# Autodesk Inventor assembly: ENSAMBLE CUERPO M 2020-9.5L
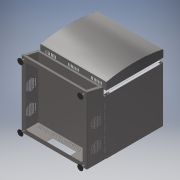
[picture p0: Inventor's stored thumbnail of the model, 180x180]
Saved by Autodesk Inventor 2017 (Build 210142000, 142)
## iProperties
Created: 2021-02-12
Part Number: ENSAMBLE CUERPO M 2020-9.5L
Description: STEP AP214
Document SubType Name: Assembly
Designer: USUARIO
Sending System: SolidWorks 2013
Preprocessor: SwSTEP 2.0
Title: ENSAMBLE CUERPO M 2020-9.5L.STEP
Revision Number: ANY
## Documents named in this file (10)
- D:\Laboratorio\Mufla\2021\Mufla 9L Psoc Artilab #0045884XX OP202139\Modelo\ENSAMBLE CUERPO M 2020-9.5L.iam
- D:\Laboratorio\Mufla\2021\Mufla 9L Psoc Artilab #0045884XX OP202139\Modelo\BASE M 2019-9.5L.ipt
- D:\Laboratorio\Mufla\2021\Mufla 9L Psoc Artilab #0045884XX OP202139\Modelo\TUERCA REMACHABLE 0,3125.ipt
- D:\Laboratorio\Mufla\2021\Mufla 9L Psoc Artilab #0045884XX OP202139\Modelo\PATA 5-16.ipt
- D:\Laboratorio\Mufla\2021\Mufla 9L Psoc Artilab #0045884XX OP202139\Modelo\RESPIRADERO M2018-2.2L.ipt
- D:\Laboratorio\Mufla\2021\Mufla 9L Psoc Artilab #0045884XX OP202139\Modelo\SEPARADOR M 2020-9.5L.ipt
- D:\Laboratorio\Mufla\2021\Mufla 9L Psoc Artilab #0045884XX OP202139\Modelo\ENSAMBLE CUERPO INTERIOR M12020-9.5L.iam
- D:\Laboratorio\Mufla\2021\Mufla 9L Psoc Artilab #0045884XX OP202139\Modelo\EnsambleAislante.iam
- D:\Laboratorio\Mufla\2021\Mufla 9L Psoc Artilab #0045884XX OP202139\Modelo\TAPA FRONTAL M 2020-9.5L.ipt
- D:\Laboratorio\Mufla\2021\Mufla 9L Psoc Artilab #0045884XX OP202139\Modelo\ENSAMBLE CUERPO PUERTA M 2020-9.5L.iam
## Components (14 placed, 14 different names)
1. BASE M 2019-9.5L_1
2. TUERCA REMACHABLE 0,3125_2
3. TUERCA REMACHABLE 0,3125_3
4. TUERCA REMACHABLE 0,3125_4
5. PATA 5-16_5
6. PATA 5-16_6
7. PATA 5-16_7
8. PATA 5-16_8
9. RESPIRADERO M2018-2.2L_9
10. SEPARADOR M 2020-9.5L_10 — Mate:1
11. ENSAMBLE CUERPO INTERIOR M12020-9.5L_11 [sub-assembly] — Flush:1, Mate:3, Flush:2, Mate:4, Mate:5, Flush:3, Flush:4
12. EnsambleAislante:1 [sub-assembly] — Mate:1, Flush:1, Mate:5
13. TAPA FRONTAL M 2020-9.5L:1 — Mate:3, Flush:2, Mate:4
14. ENSAMBLE CUERPO PUERTA M 2020-9.5L:1 [sub-assembly] — Flush:3, Flush:4
## Relationships (8: Mate 4, Flush 4)
- Mate:1: SEPARADOR M 2020-9.5L_10 ↔ EnsambleAislante:1
- Flush:1: ENSAMBLE CUERPO INTERIOR M12020-9.5L_11 ↔ EnsambleAislante:1
- Mate:3 (1 mm): ENSAMBLE CUERPO INTERIOR M12020-9.5L_11 ↔ TAPA FRONTAL M 2020-9.5L:1
- Flush:2: ENSAMBLE CUERPO INTERIOR M12020-9.5L_11 ↔ TAPA FRONTAL M 2020-9.5L:1
- Mate:4 (1 mm): ENSAMBLE CUERPO INTERIOR M12020-9.5L_11 ↔ TAPA FRONTAL M 2020-9.5L:1
- Mate:5: ENSAMBLE CUERPO INTERIOR M12020-9.5L_11 ↔ EnsambleAislante:1
- Flush:3: ENSAMBLE CUERPO INTERIOR M12020-9.5L_11 ↔ ENSAMBLE CUERPO PUERTA M 2020-9.5L:1
- Flush:4: ENSAMBLE CUERPO INTERIOR M12020-9.5L_11 ↔ ENSAMBLE CUERPO PUERTA M 2020-9.5L:1
